# Autodesk Inventor assembly: wheelchair_secure_devices
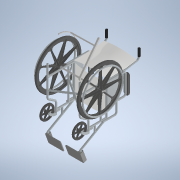
[picture p0: Inventor's stored thumbnail of the model, 180x180]
Saved by Autodesk Inventor 2021 (Build 250183000, 183)
## iProperties
Created: 2021-05-28
Part Number: wheelchair_secure_devices
Document SubType Name: Assembly
## Documents named in this file (6)
- C:\Users\ocon0143\OneDrive - Flinders\Advn Mech Design Shared\6_Development\2_Design\inventor\securing_mechanism\wheelchair_secure_devices.iam
- C:\Users\ocon0143\OneDrive - Flinders\Advn Mech Design Shared\6_Development\2_Design\inventor\securing_mechanism\secure_arm_holder.ipt
- C:\Users\ocon0143\OneDrive - Flinders\Advn Mech Design Shared\6_Development\2_Design\inventor\securing_mechanism\secure_wheel_bar.ipt
- C:\Users\ocon0143\OneDrive - Flinders\Advn Mech Design Shared\6_Development\2_Design\inventor\securing_mechanism\secure_width_bar.ipt
- C:\Users\ocon0143\OneDrive - Flinders\Advn Mech Design Shared\6_Development\2_Design\inventor\vehicle_wheelchair\wheelchair\wheelchair.ipt
- C:\Users\ocon0143\OneDrive - Flinders\Advn Mech Design Shared\6_Development\2_Design\inventor\securing_mechanism\axle_example.ipt
## Components (5 placed, 5 different names)
1. secure_arm_holder:1 — Mate:2
2. secure_wheel_bar:1
3. secure_width_bar:1
4. wheelchair:1 — Mate:1, Flush:1
5. axle_example:1 — Mate:1, Flush:2, Mate:2
## Relationships (4: Mate 2, Flush 2)
- Mate:1: wheelchair:1 ↔ axle_example:1
- Flush:1 (220 mm): wheelchair:1
- Flush:2: axle_example:1
- Mate:2: secure_arm_holder:1 ↔ axle_example:1
